# Autodesk Inventor assembly: SHOOT CAD FINAL
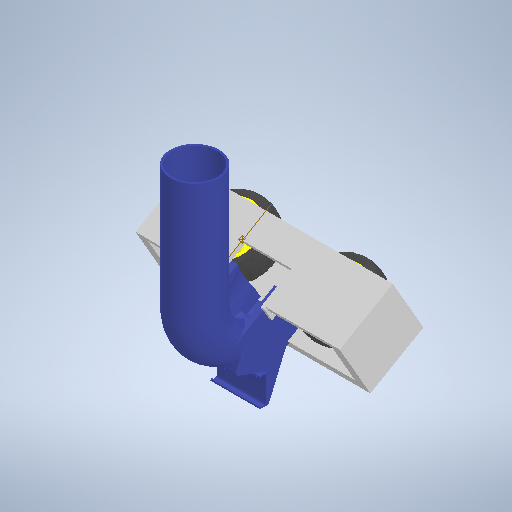
[picture p0: Inventor's stored thumbnail of the model, 512x512]
Saved by Autodesk Inventor 2025.3 (Build 293356000, 356)
## iProperties
Created: 2026-04-17
Part Number: SHOOT CAD FINAL
Document SubType Name: Assembly
Designer: lenovo
Author: lenovo
## Documents named in this file (6)
- C:\Users\lenovo\OneDrive\Desktop\BASICS PROJECT\BASICS SHOOT CAD\SHOOT CAD FINAL.iam
- C:\Users\lenovo\OneDrive\Desktop\BASICS PROJECT\shooting\my parts\Container Tube v2.ipt
- C:\Users\lenovo\OneDrive\Desktop\BASICS PROJECT\shooting\my parts\upper part shooter.ipt
- C:\Users\lenovo\OneDrive\Desktop\BASICS PROJECT\shooting\my parts\shaft shooting.ipt
- C:\Users\lenovo\OneDrive\Desktop\BASICS PROJECT\shooting\my parts\Wheel.ipt
- C:\Users\lenovo\OneDrive\Desktop\BASICS PROJECT\BASICS SHOOT CAD\Motor12v.iam
## Components (8 placed, 5 different names)
1. Container Tube v2:1 — Mate:1, Mate:2, Mate:3
2. upper part shooter:1 — Mate:1, Mate:2, Mate:3, Mate:12, Mate:13, Mate:14
3. shaft shooting:1 — Mate:6, Mate:7, Mate:10, Mate:11, Mate:14
4. shaft shooting:2 — Mate:4, Mate:5, Mate:8, Mate:9, Mate:12
5. Wheel:1 — Mate:4, Mate:5
6. Wheel:2 — Mate:6, Mate:7
7. Motor12v:1 [sub-assembly] — Mate:8, Mate:9, Mate:13
8. Motor12v:2 [sub-assembly] — Mate:10, Mate:11
## Relationships (14: Mate 14)
- Mate:1: Container Tube v2:1 ↔ upper part shooter:1
- Mate:2: Container Tube v2:1 ↔ upper part shooter:1
- Mate:3: Container Tube v2:1 ↔ upper part shooter:1
- Mate:4: shaft shooting:2 ↔ Wheel:1
- Mate:5: shaft shooting:2 ↔ Wheel:1
- Mate:6: shaft shooting:1 ↔ Wheel:2
- Mate:7: shaft shooting:1 ↔ Wheel:2
- Mate:8: shaft shooting:2 ↔ Motor12v:1
- Mate:9: shaft shooting:2 ↔ Motor12v:1
- Mate:10: shaft shooting:1 ↔ Motor12v:2
- Mate:11: shaft shooting:1 ↔ Motor12v:2
- Mate:12: upper part shooter:1 ↔ shaft shooting:2
- Mate:13: upper part shooter:1 ↔ Motor12v:1
- Mate:14: upper part shooter:1 ↔ shaft shooting:1
